# Autodesk Inventor assembly: MAIN Gripper assembly 2018
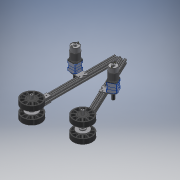
[picture p0: Inventor's stored thumbnail of the model, 180x180]
Saved by Autodesk Inventor 2018 (Build 220112000, 112)
## iProperties
Created: 2019-01-23
Part Number: MAIN Gripper assembly 2018
Document SubType Name: Assembly
Designer: s-2513225
Author: s-2513225
## Documents named in this file (4)
- E:\Robotics\ball intake 2018\MAIN Gripper assembly 2018.iam
- E:\Robotics\ball intake 2018\Left arm.iam
- E:\Robotics\ball intake 2018\right arm.iam
- E:\Robotics\ball intake 2018\hinge.ipt
## Components (4 placed, 3 different names)
1. Left arm:1 [sub-assembly] — Flush:1, Mate:1, Flush:2
2. right arm:1 [sub-assembly] — Flush:3, Flush:4, Mate:2
3. hinge:1 — Flush:1, Mate:1, Flush:2, Mate:4, Mate:5
4. hinge:2 — Flush:3, Flush:4, Mate:2, Mate:4, Mate:5
## Relationships (8: Flush 4, Mate 4)
- Flush:1: Left arm:1 ↔ hinge:1
- Mate:1: Left arm:1 ↔ hinge:1
- Flush:2: Left arm:1 ↔ hinge:1
- Flush:3: right arm:1 ↔ hinge:2
- Flush:4: right arm:1 ↔ hinge:2
- Mate:2: right arm:1 ↔ hinge:2
- Mate:4: hinge:1 ↔ hinge:2
- Mate:5: hinge:1 ↔ hinge:2
